# Autodesk Inventor assembly: ASY MSC 900.6 BASE FRAME
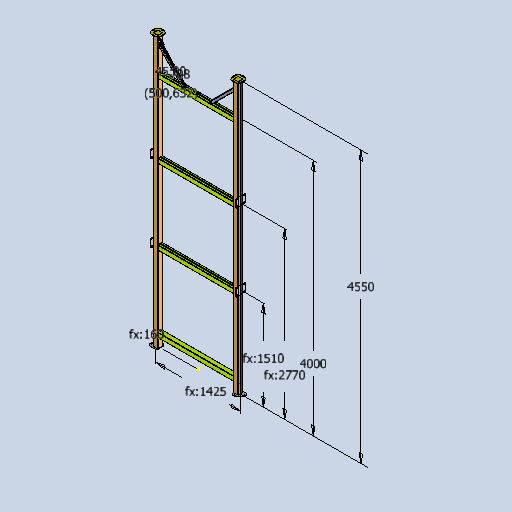
[picture p0: Inventor's stored thumbnail of the model, 512x512]
Saved by Autodesk Inventor 2025 (Build 290162010, 162A)
## iProperties
_SolveAssemblyDoc: Frame Generator Solve Assembly
_Version: 25.0.0
Created: 2024-06-30
Part Number: ASY MSC 900.6 BASE FRAME
Document SubType Name: Assembly
Designer: pokla
Stock Number: МОО 900.6 базовая рама 3
Author: pokla
## Documents named in this file (6)
- C:\Users\admin\YandexDisk-badmisterfox\домашниий пк\Inventor\Manturovo\Manturovo_Se-clar\Pillars\ASY MSC 900.6 base frame.iam
- C:\Users\admin\YandexDisk-badmisterfox\домашниий пк\Inventor\Manturovo\Manturovo_Se-clar\Pillars\MSC DIM 009.6 base frame sketch.ipt
- C:\Users\admin\YandexDisk-badmisterfox\домашниий пк\Inventor\Manturovo\Manturovo_Se-clar\Pillars\ASY MSC 900.6.1 base frame.iam
- C:\Users\admin\YandexDisk-badmisterfox\домашниий пк\Inventor\Manturovo\Manturovo_Se-clar\MSC 902 flange frame heel.ipt
- C:\Users\admin\YandexDisk-badmisterfox\домашниий пк\Inventor\Manturovo\Manturovo_Se-clar\MSC 906 flange frame.ipt
- C:\Users\admin\YandexDisk-badmisterfox\домашниий пк\Inventor\Manturovo\Manturovo_Se-clar\MSC 908 transverse pillar plate.ipt
## Components (10 placed, 5 different names)
1. MSC DIM 009.6 base frame sketch.ipt:1
2. ASY MSC 900.6.1 base frame.iam:1 [sub-assembly] — Rigid:3, Rigid:4, Rigid:5, Rigid:6, Mate:1, Mate:3, Mate:4, Flush:1
3. MSC 902 flange frame heel.ipt:1 — Rigid:5, Mate:2, Mate:5
4. MSC 902 flange frame heel.ipt:2 — Rigid:6
5. MSC 906 flange frame.ipt:1 — Rigid:3
6. MSC 906 flange frame.ipt:2 — Rigid:4
7. MSC 908 transverse pillar plate.ipt:1 — Mate:1, Mate:2, Mate:3, Rigid:11
8. MSC 908 transverse pillar plate.ipt:2 — Mate:4, Mate:5, Flush:1, Rigid:12
9. MSC 908 transverse pillar plate.ipt:3 — Rigid:11
10. MSC 908 transverse pillar plate.ipt:4 — Rigid:12
## Relationships (12: WeldJoint 6, Mate 5, Flush 1)
- Rigid:3 [WeldJoint]: ASY MSC 900.6.1 base frame.iam:1 ↔ MSC 906 flange frame.ipt:1
- Rigid:4 [WeldJoint]: ASY MSC 900.6.1 base frame.iam:1 ↔ MSC 906 flange frame.ipt:2
- Rigid:5 [WeldJoint]: ASY MSC 900.6.1 base frame.iam:1 ↔ MSC 902 flange frame heel.ipt:1
- Rigid:6 [WeldJoint]: ASY MSC 900.6.1 base frame.iam:1 ↔ MSC 902 flange frame heel.ipt:2
- Mate:1: ASY MSC 900.6.1 base frame.iam:1 ↔ MSC 908 transverse pillar plate.ipt:1
- Mate:2 (2736 mm): MSC 902 flange frame heel.ipt:1 ↔ MSC 908 transverse pillar plate.ipt:1
- Mate:3: ASY MSC 900.6.1 base frame.iam:1 ↔ MSC 908 transverse pillar plate.ipt:1
- Rigid:11 [WeldJoint] (1425 mm): MSC 908 transverse pillar plate.ipt:1 ↔ MSC 908 transverse pillar plate.ipt:3
- Mate:4: ASY MSC 900.6.1 base frame.iam:1 ↔ MSC 908 transverse pillar plate.ipt:2
- Mate:5 (1446 mm): MSC 902 flange frame heel.ipt:1 ↔ MSC 908 transverse pillar plate.ipt:2
- Flush:1: ASY MSC 900.6.1 base frame.iam:1 ↔ MSC 908 transverse pillar plate.ipt:2
- Rigid:12 [WeldJoint] (1425 mm): MSC 908 transverse pillar plate.ipt:2 ↔ MSC 908 transverse pillar plate.ipt:4
